# Autodesk Inventor assembly: spur1
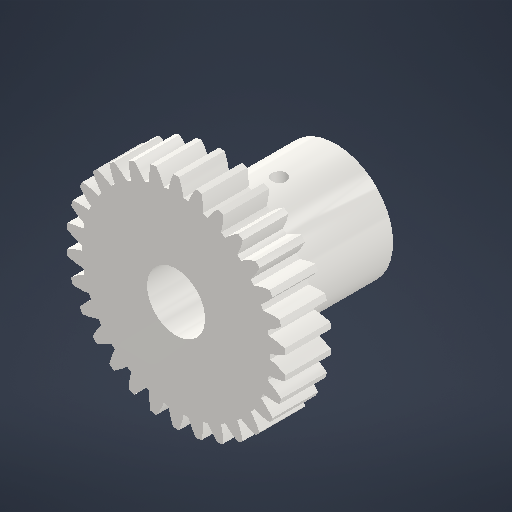
[picture p0: Inventor's stored thumbnail of the model, 512x512]
Saved by Autodesk Inventor 2026.1 (Build 301233000, 233)
## iProperties
Created: 2025-11-11
Part Number: spur1
Document SubType Name: Assembly
Designer: Mukund Advaith
Author: Mukund Advaith
## Documents named in this file (2)
- C:\Users\mukun\Downloads\project\finalreport\spur1.iam
- C:\Users\mukun\Downloads\project\finalreport\spur1\Design Accelerator\Spur Gears2.iam
## Components (1 placed, 1 different names)
1. Spur Gears:1 [sub-assembly] — Flush:1, Flush:2, Flush:3
## Relationships (3: Flush 3)
- Flush:1: Spur Gears:1
- Flush:2: Spur Gears:1
- Flush:3: Spur Gears:1
